# Autodesk Inventor assembly: Quadro_Eletrico_Trituradora
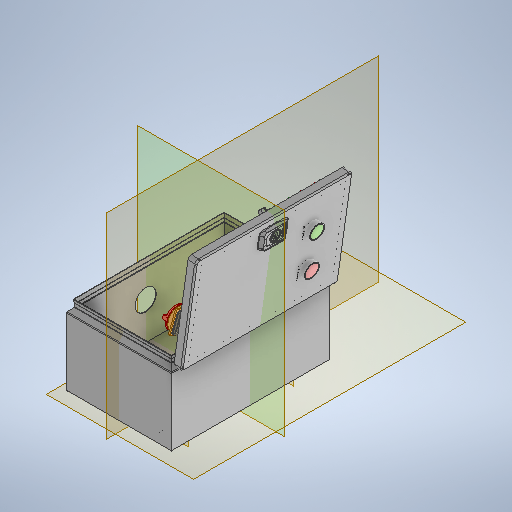
[picture p0: Inventor's stored thumbnail of the model, 512x512]
Saved by Autodesk Inventor 2025.2 (Build 292293000, 293)
## iProperties
Category: PARTsolutions
Company: RITTAL
Created: 2025-05-02
Part Number: Quadro_Eletrico_Trituradora
Catalog Web Link: www.cadenas.de
Description: KX E-Box-stainless steel
Vendor: RITTAL
Document SubType Name: Assembly
Designer: psAdmin
Manufacturer: RITTAL
Mass: 539.801 g
Surface Area: 7071.18 cm^2
Volume: 539.801 cm^3
Density: 1 g/cm^3
PSOL_IDENT_0: {$CADENAS_DATA/23d-libs/rittal/schaltschranksys/edelstahl/kleingehause/eb_edel_2_0_asmtab.prj},188 {
PSOL_IDENT_1: VTYP=3D},{STYP=ASSTAB},{NB=1301.000(1)},{LINA=1301.000},{NN=KX E-Box},{DATE=28.04.2025 21:10:46},{GE
PSOL_IDENT_2: OMDATE=11.04.2025 11:21:28},{VERSION=},{LINEID=690},{WBVAR=DETAIL},{WBNUMERIC=DETAIL}  {NB=1301.000(
PSOL_IDENT_3: 1)},{LINA=1301.000},{KT=DUMMY},{BEST=1301.000},{INFOPAGE=-},{DETAIL=1},{INFOWWW=Website},{BEZ1=KX El
PSOL_IDENT_4: ektronik-Box},{BEZ2=Edelstahl, 1.4404},{BEZ3=eintürig},{B=200},{H=300},{T=155},{F=175},{G=285},{GEW=
PSOL_IDENT_5: 3,889},{INFOPATH=http://www.rittal.com/com-en/part/1301000},{CNSECLASS51=27-18-01-02},{CNSECLASS70=2
PSOL_IDENT_6: 7-18-01-01},{CNSECLASS80=27-18-01-01},{CNSETIM40=EC002713},{PPATH=assemblies_eb_edel_2_0/kx_eb_edel_
PSOL_IDENT_7: new_asmtpl.prj},{BESTE1=1301},{BESTE2=000},{CNSETIM80=EC000261},{CNSETIM90=EC000261},{CNSECLASS60=27
PSOL_IDENT_8: -18-01-01},{UNSPSC=31-26-15-02}
NB: 1301.000(1)
NN: KX E-Box
NT: stainless steel
NBSYN: $BEST.($DETAIL.)
LINA: 1301.000
CATALOG: Rittal
BEST: 1301.000
DETAIL: high
INFOWWW: Website
BEZ1: KX E-Box
BEZ2: Stainless steel, 1.4404
BEZ3: single door
B: 200
H: 300
T: 155
F: 175
G: 285
CNSECLASS70: 27-18-01-01
CNSECLASS80: 27-18-01-01
CNSETIM80: EC000261
CNSETIM90: EC000261
CNSECLASS60: 27-18-01-01
UNSPSC: 31-26-15-02
SUPPLIER: RITTAL
ARTICLENO: 1301.000(1)
BOMINFO: 1301.000
CREATOR: CADENAS GmbH
Title: 1301.000
Author: Cadenas PARTsolutions
Comments: stainless steel
## Documents named in this file (15)
- C:\Users\ishad\OneDrive\Desktop\Quadro eletrico trituradora\AIS2024\1301_000_1_\Quadro_Eletrico_Trituradora.iam
- C:\Users\ishad\OneDrive\Desktop\Quadro eletrico trituradora\AIS2024\1301_000_1_\1301_000_1_(1).ipt
- C:\Users\ishad\OneDrive\Desktop\Quadro eletrico trituradora\AIS2024\1301_000_1_\1301_000_6_(1).ipt
- C:\Users\ishad\OneDrive\Desktop\Quadro eletrico trituradora\AIS2024\1301_000_1_\1301_000_4_(1).ipt
- C:\Users\ishad\OneDrive\Desktop\Quadro eletrico trituradora\AIS2024\1301_000_1_\1301_000_2_(1).ipt
- C:\Users\ishad\OneDrive\Desktop\Quadro eletrico trituradora\AIS2024\1301_000_1_\1301_000_5_(1).ipt
- C:\Users\ishad\OneDrive\Desktop\Quadro eletrico trituradora\AIS2024\1301_000_1_\1301_000_3_(1).ipt
- C:\Users\ishad\OneDrive\Desktop\Quadro eletrico trituradora\AIS2024\1301_000_1_\1301_000_10_(1).ipt
- C:\Users\ishad\OneDrive\Desktop\Quadro eletrico trituradora\AIS2024\1301_000_1_\PP0735H(1).ipt
- C:\Users\ishad\OneDrive\Desktop\Quadro eletrico trituradora\AIS2024\1301_000_1_\Light Stack.ipt
- C:\Users\ishad\OneDrive\Desktop\Quadro eletrico trituradora\AIS2024\1301_000_1_\3-phase CB\3-phase CB\3-phase CB.ipt
- C:\Users\ishad\OneDrive\Desktop\Quadro eletrico trituradora\AIS2024\1301_000_1_\3RV1011-1EA10\3RV1011-1EA10\3RV1011-1EA10.ipt
- C:\Users\ishad\OneDrive\Desktop\Quadro eletrico trituradora\AIS2024\1301_000_1_\Eaton main switch P1-25-M4-SVB - switch\Eaton main switch P1-25-M4-SVB - switch\Eaton main switch P1-25-M4-SVB - switch.ipt
- C:\Users\ishad\OneDrive\Desktop\Quadro eletrico trituradora\AIS2024\1301_000_1_\XB2-BA42\XB2-BA42\XB2-BA42.ipt
- C:\Users\ishad\OneDrive\Desktop\Quadro eletrico trituradora\AIS2024\1301_000_1_\XB2-BA31\XB2-BA31\XB2-BA31.ipt
## Components (21 placed, 14 different names)
1. 1301_000_1_(1):1 — to_MP_XY@1 <-> MONTAGEPLATTE_XY@2, to_MP_Z@1 <-> MONTAGEPLATTE_Z@2, to_MP_YZ@1 <-> MONTAGEPLATTE_YZ@2, to_HINGE_1_XY@1 <-> HINGE_XY@3, to_HINGE_1_Z@1 <-> HINGE_Z@3, to_HINGE_1_YZ@1 <-> HINGE_YZ@3, to_HINGE_2_XY@1 <-> HINGE_XY@4, to_HINGE_2_Z@1 <-> HINGE_Z@4, to_HINGE_2_YZ@1 <-> HINGE_YZ@4, to_L_Winkel_Bottom_XY@1 <-> SEITENTEIL_XY@7, to_L_Winkel_Bottom_Z@1 <-> SEITENTEIL_Z@7, to_L_Winkel_Bottom_YZ@1 <-> SEITENTEIL_YZ@7, to_L_Winkel_Top_XY@1 <-> SEITENTEIL_XY@10, to_L_Winkel_Top_Z@1 <-> SEITENTEIL_Z@10, to_L_Winkel_Top_YZ@1 <-> SEITENTEIL_YZ@10, Angle:11, Mate:29, Mate:44, Mate:45, Mate:46, Mate:47, Mate:48, Mate:49, Mate:50, Mate:51, Mate:52, Mate:53, Mate:54, Mate:55, Mate:56, Mate:57
2. 1301_000_6_(1):1 — to_MP_XY@1 <-> MONTAGEPLATTE_XY@2, to_MP_Z@1 <-> MONTAGEPLATTE_Z@2, to_MP_YZ@1 <-> MONTAGEPLATTE_YZ@2, Mate:23, Mate:24, Mate:30, Mate:31, Mate:36, Mate:37
3. 1301_000_4_(1):1 — to_HINGE_1_XY@1 <-> HINGE_XY@3, to_HINGE_1_Z@1 <-> HINGE_Z@3, to_HINGE_1_YZ@1 <-> HINGE_YZ@3
4. 1301_000_4_(1):2 — to_HINGE_2_XY@1 <-> HINGE_XY@4, to_HINGE_2_Z@1 <-> HINGE_Z@4, to_HINGE_2_YZ@1 <-> HINGE_YZ@4, DECKEL_XY@4 <-> to_HINGE_1_XY@5, DECKEL_Z@4 <-> to_HINGE_1_Z@5
5. 1301_000_2_(1):1 — DECKEL_XY@4 <-> to_HINGE_1_XY@5, DECKEL_Z@4 <-> to_HINGE_1_Z@5, VB_XY@5 <-> VV_XY@6, VB_Z@5 <-> VV_Z@6, VB_YZ@5 <-> VV_YZ@6, Mate:58, Mate:59, Mate:60, Mate:61, Mate:62, Mate:63
6. 1301_000_5_(1):1 — VB_XY@5 <-> VV_XY@6, VB_Z@5 <-> VV_Z@6, VB_YZ@5 <-> VV_YZ@6
7. 1301_000_3_(1):1 — to_L_Winkel_Bottom_XY@1 <-> SEITENTEIL_XY@7, to_L_Winkel_Bottom_Z@1 <-> SEITENTEIL_Z@7, to_L_Winkel_Bottom_YZ@1 <-> SEITENTEIL_YZ@7, SC1_XY@7 <-> SCHRAUBE_XY@8, SC1_Z@7 <-> SCHRAUBE_Z@8, SC1_YZ@7 <-> SCHRAUBE_YZ@8, SC2_XY@7 <-> SCHRAUBE_XY@9, SC2_Z@7 <-> SCHRAUBE_Z@9, SC2_YZ@7 <-> SCHRAUBE_YZ@9
8. 1301_000_10_(1):1 — SC1_XY@7 <-> SCHRAUBE_XY@8, SC1_Z@7 <-> SCHRAUBE_Z@8, SC1_YZ@7 <-> SCHRAUBE_YZ@8
9. 1301_000_10_(1):2 — SC2_XY@7 <-> SCHRAUBE_XY@9, SC2_Z@7 <-> SCHRAUBE_Z@9, SC2_YZ@7 <-> SCHRAUBE_YZ@9
10. 1301_000_3_(1):2 — to_L_Winkel_Top_XY@1 <-> SEITENTEIL_XY@10, to_L_Winkel_Top_Z@1 <-> SEITENTEIL_Z@10, to_L_Winkel_Top_YZ@1 <-> SEITENTEIL_YZ@10, SC1_XY@10 <-> SCHRAUBE_XY@11, SC1_Z@10 <-> SCHRAUBE_Z@11, SC1_YZ@10 <-> SCHRAUBE_YZ@11, SC2_XY@10 <-> SCHRAUBE_XY@12, SC2_Z@10 <-> SCHRAUBE_Z@12, SC2_YZ@10 <-> SCHRAUBE_YZ@12
11. 1301_000_10_(1):3 — SC1_XY@10 <-> SCHRAUBE_XY@11, SC1_Z@10 <-> SCHRAUBE_Z@11, SC1_YZ@10 <-> SCHRAUBE_YZ@11
12. 1301_000_10_(1):4 — SC2_XY@10 <-> SCHRAUBE_XY@12, SC2_Z@10 <-> SCHRAUBE_Z@12, SC2_YZ@10 <-> SCHRAUBE_YZ@12
13. PP0735H(1):1 — Mate:24, Mate:31, Mate:37
14. PP0735H(1):2 — Mate:23, Mate:30, Mate:36, Mate:38, Mate:39, Mate:40, Mate:41, Mate:43
15. Light Stack:1 — Angle:11, Mate:29
16. 3-phase CB:1 — Mate:38, Mate:39
17. 3RV1011-1EA10:1 — Mate:40, Mate:41, Mate:42
18. 3RV1011-1EA10:2 — Mate:42, Mate:43
19. Eaton main switch P1-25-M4-SVB - switch:1 — Mate:44, Mate:45, Mate:46, Mate:47, Mate:48, Mate:49, Mate:50, Mate:51, Mate:52, Mate:53, Mate:54, Mate:55, Mate:56, Mate:57
20. XB2-BA31:1 — Mate:58, Mate:59, Mate:62
21. XB2-BA42:1 — Mate:60, Mate:61, Mate:63
## Relationships (66: Mate 55, Angle 11)
- to_MP_XY@1 <-> MONTAGEPLATTE_XY@2 [Mate]: 1301_000_1_(1):1 ↔ 1301_000_6_(1):1
- to_MP_Z@1 <-> MONTAGEPLATTE_Z@2 [Mate]: 1301_000_1_(1):1 ↔ 1301_000_6_(1):1
- to_MP_YZ@1 <-> MONTAGEPLATTE_YZ@2 [Angle] (0 deg): 1301_000_1_(1):1 ↔ 1301_000_6_(1):1
- to_HINGE_1_XY@1 <-> HINGE_XY@3 [Mate]: 1301_000_1_(1):1 ↔ 1301_000_4_(1):1
- to_HINGE_1_Z@1 <-> HINGE_Z@3 [Mate]: 1301_000_1_(1):1 ↔ 1301_000_4_(1):1
- to_HINGE_1_YZ@1 <-> HINGE_YZ@3 [Angle] (90 deg): 1301_000_1_(1):1 ↔ 1301_000_4_(1):1
- to_HINGE_2_XY@1 <-> HINGE_XY@4 [Mate]: 1301_000_1_(1):1 ↔ 1301_000_4_(1):2
- to_HINGE_2_Z@1 <-> HINGE_Z@4 [Mate]: 1301_000_1_(1):1 ↔ 1301_000_4_(1):2
- to_HINGE_2_YZ@1 <-> HINGE_YZ@4 [Angle] (90 deg): 1301_000_1_(1):1 ↔ 1301_000_4_(1):2
- DECKEL_XY@4 <-> to_HINGE_1_XY@5 [Mate]: 1301_000_4_(1):2 ↔ 1301_000_2_(1):1
- DECKEL_Z@4 <-> to_HINGE_1_Z@5 [Mate]: 1301_000_4_(1):2 ↔ 1301_000_2_(1):1
- VB_XY@5 <-> VV_XY@6 [Mate]: 1301_000_2_(1):1 ↔ 1301_000_5_(1):1
- VB_Z@5 <-> VV_Z@6 [Mate]: 1301_000_2_(1):1 ↔ 1301_000_5_(1):1
- VB_YZ@5 <-> VV_YZ@6 [Angle] (0 deg): 1301_000_2_(1):1 ↔ 1301_000_5_(1):1
- to_L_Winkel_Bottom_XY@1 <-> SEITENTEIL_XY@7 [Mate] (-0.25 mm): 1301_000_1_(1):1 ↔ 1301_000_3_(1):1
- to_L_Winkel_Bottom_Z@1 <-> SEITENTEIL_Z@7 [Mate]: 1301_000_1_(1):1 ↔ 1301_000_3_(1):1
- to_L_Winkel_Bottom_YZ@1 <-> SEITENTEIL_YZ@7 [Angle] (-90 deg): 1301_000_1_(1):1 ↔ 1301_000_3_(1):1
- SC1_XY@7 <-> SCHRAUBE_XY@8 [Mate] (-1.575 mm): 1301_000_3_(1):1 ↔ 1301_000_10_(1):1
- SC1_Z@7 <-> SCHRAUBE_Z@8 [Mate]: 1301_000_3_(1):1 ↔ 1301_000_10_(1):1
- SC1_YZ@7 <-> SCHRAUBE_YZ@8 [Angle] (0 deg): 1301_000_3_(1):1 ↔ 1301_000_10_(1):1
- SC2_XY@7 <-> SCHRAUBE_XY@9 [Mate] (-1.575 mm): 1301_000_3_(1):1 ↔ 1301_000_10_(1):2
- SC2_Z@7 <-> SCHRAUBE_Z@9 [Mate]: 1301_000_3_(1):1 ↔ 1301_000_10_(1):2
- SC2_YZ@7 <-> SCHRAUBE_YZ@9 [Angle] (0 deg): 1301_000_3_(1):1 ↔ 1301_000_10_(1):2
- to_L_Winkel_Top_XY@1 <-> SEITENTEIL_XY@10 [Mate] (-0.25 mm): 1301_000_1_(1):1 ↔ 1301_000_3_(1):2
- to_L_Winkel_Top_Z@1 <-> SEITENTEIL_Z@10 [Mate]: 1301_000_1_(1):1 ↔ 1301_000_3_(1):2
- to_L_Winkel_Top_YZ@1 <-> SEITENTEIL_YZ@10 [Angle] (90 deg): 1301_000_1_(1):1 ↔ 1301_000_3_(1):2
- SC1_XY@10 <-> SCHRAUBE_XY@11 [Mate] (-1.575 mm): 1301_000_3_(1):2 ↔ 1301_000_10_(1):3
- SC1_Z@10 <-> SCHRAUBE_Z@11 [Mate]: 1301_000_3_(1):2 ↔ 1301_000_10_(1):3
- SC1_YZ@10 <-> SCHRAUBE_YZ@11 [Angle] (0 deg): 1301_000_3_(1):2 ↔ 1301_000_10_(1):3
- SC2_XY@10 <-> SCHRAUBE_XY@12 [Mate] (-1.575 mm): 1301_000_3_(1):2 ↔ 1301_000_10_(1):4
- SC2_Z@10 <-> SCHRAUBE_Z@12 [Mate]: 1301_000_3_(1):2 ↔ 1301_000_10_(1):4
- SC2_YZ@10 <-> SCHRAUBE_YZ@12 [Angle] (0 deg): 1301_000_3_(1):2 ↔ 1301_000_10_(1):4
- Mate:23: 1301_000_6_(1):1 ↔ PP0735H(1):2
- Mate:24: 1301_000_6_(1):1 ↔ PP0735H(1):1
- Angle:11 (180 deg): 1301_000_1_(1):1 ↔ Light Stack:1
- Mate:29: 1301_000_1_(1):1 ↔ Light Stack:1
- Mate:30: 1301_000_6_(1):1 ↔ PP0735H(1):2
- Mate:31: 1301_000_6_(1):1 ↔ PP0735H(1):1
- Mate:36 (0.8 mm): 1301_000_6_(1):1 ↔ PP0735H(1):2
- Mate:37 (0.8 mm): 1301_000_6_(1):1 ↔ PP0735H(1):1
- Mate:38: PP0735H(1):2 ↔ 3-phase CB:1
- Mate:39: PP0735H(1):2 ↔ 3-phase CB:1
- Mate:40: PP0735H(1):2 ↔ 3RV1011-1EA10:1
- Mate:41: PP0735H(1):2 ↔ 3RV1011-1EA10:1
- Mate:42: 3RV1011-1EA10:1 ↔ 3RV1011-1EA10:2
- Mate:43: PP0735H(1):2 ↔ 3RV1011-1EA10:2
- Mate:44: 1301_000_1_(1):1 ↔ Eaton main switch P1-25-M4-SVB - switch:1
- Mate:45: 1301_000_1_(1):1 ↔ Eaton main switch P1-25-M4-SVB - switch:1
- Mate:46: 1301_000_1_(1):1 ↔ Eaton main switch P1-25-M4-SVB - switch:1
- Mate:47: 1301_000_1_(1):1 ↔ Eaton main switch P1-25-M4-SVB - switch:1
- Mate:48: 1301_000_1_(1):1 ↔ Eaton main switch P1-25-M4-SVB - switch:1
- Mate:49: 1301_000_1_(1):1 ↔ Eaton main switch P1-25-M4-SVB - switch:1
- Mate:50: 1301_000_1_(1):1 ↔ Eaton main switch P1-25-M4-SVB - switch:1
- Mate:51: 1301_000_1_(1):1 ↔ Eaton main switch P1-25-M4-SVB - switch:1
- Mate:52: 1301_000_1_(1):1 ↔ Eaton main switch P1-25-M4-SVB - switch:1
- Mate:53: 1301_000_1_(1):1 ↔ Eaton main switch P1-25-M4-SVB - switch:1
- Mate:54: 1301_000_1_(1):1 ↔ Eaton main switch P1-25-M4-SVB - switch:1
- Mate:55: 1301_000_1_(1):1 ↔ Eaton main switch P1-25-M4-SVB - switch:1
- Mate:56: 1301_000_1_(1):1 ↔ Eaton main switch P1-25-M4-SVB - switch:1
- Mate:57: 1301_000_1_(1):1 ↔ Eaton main switch P1-25-M4-SVB - switch:1
- Mate:58: 1301_000_2_(1):1 ↔ XB2-BA31:1
- Mate:59: 1301_000_2_(1):1 ↔ XB2-BA31:1
- Mate:60: 1301_000_2_(1):1 ↔ XB2-BA42:1
- Mate:61: 1301_000_2_(1):1 ↔ XB2-BA42:1
- Mate:62: 1301_000_2_(1):1 ↔ XB2-BA31:1
- Mate:63: 1301_000_2_(1):1 ↔ XB2-BA42:1
